# Autodesk Inventor assembly: TrussCC_printasm
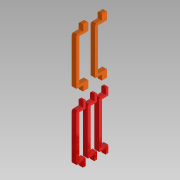
[picture p0: Inventor's stored thumbnail of the model, 180x180]
Saved by Autodesk Inventor 2021 (Build 250183000, 183)
## iProperties
Created: 2021-02-11
Part Number: TrussCC_printasm
Document SubType Name: Assembly
Designer: kumagai
Author: kumagai
## Documents named in this file (3)
- X:\Develop\CAD\PlaRails\TrussCC_printasm.iam
- X:\Develop\CAD\PlaRails\TrussCC_S1.ipt
- X:\Develop\CAD\PlaRails\TrussCC_S2.ipt
## Components (5 placed, 2 different names)
1. TrussCC_S1:1 — フラッシュ:1, フラッシュ:2, フラッシュ:3
2. TrussCC_S1:2
3. TrussCC_S1:3
4. TrussCC_S2:1 — フラッシュ:1, フラッシュ:2, フラッシュ:3
5. TrussCC_S2:2
## Component patterns: (3 elements, first: TrussCC_S1:1), (2 elements, first: TrussCC_S2:1)
## Relationships (3: Flush 3)
- フラッシュ:1 [Flush]: TrussCC_S1:1 ↔ TrussCC_S2:1
- フラッシュ:2 [Flush] (70 mm): TrussCC_S1:1 ↔ TrussCC_S2:1
- フラッシュ:3 [Flush]: TrussCC_S1:1 ↔ TrussCC_S2:1
